# Autodesk Inventor assembly: AssembledCube
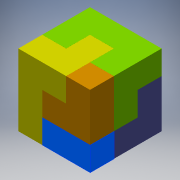
[picture p0: Inventor's stored thumbnail of the model, 180x180]
Saved by Autodesk Inventor 2019 (Build 230136000, 136)
## iProperties
Created: 2018-12-10
Part Number: AssembledCube
Document SubType Name: Assembly
Designer: Mihir
Author: Mihir
## Documents named in this file (6)
- C:\Users\Mihir\Documents\Inventor\AssembledCube.iam
- C:\Users\Mihir\Documents\Inventor\BluePiece.ipt
- C:\Users\Mihir\Documents\Inventor\GreenPiece.ipt
- C:\Users\Mihir\Documents\Inventor\OrangePiece.ipt
- C:\Users\Mihir\Documents\Inventor\PurplePiece.ipt
- C:\Users\Mihir\Documents\Inventor\YellowPiece.ipt
## Components (5 placed, 5 different names)
1. BluePiece:1 — Mate:2, Flush:3, Flush:4, Mate:3, Mate:4, Mate:7
2. GreenPiece:1 — Mate:6, Flush:6, Flush:7
3. OrangePiece:1 — Mate:1, Flush:1, Flush:2, Flush:5, Mate:5, Flush:7
4. PurplePiece:1 — Mate:1, Flush:1, Flush:2, Mate:2, Flush:3, Flush:4, Mate:6, Flush:6
5. YellowPiece:1 — Mate:3, Mate:4, Flush:5, Mate:5, Mate:7
## Relationships (14: Mate 7, Flush 7)
- Mate:1: OrangePiece:1 ↔ PurplePiece:1
- Flush:1: OrangePiece:1 ↔ PurplePiece:1
- Flush:2: OrangePiece:1 ↔ PurplePiece:1
- Mate:2: BluePiece:1 ↔ PurplePiece:1
- Flush:3: BluePiece:1 ↔ PurplePiece:1
- Flush:4: BluePiece:1 ↔ PurplePiece:1
- Mate:3: BluePiece:1 ↔ YellowPiece:1
- Mate:4: BluePiece:1 ↔ YellowPiece:1
- Flush:5: OrangePiece:1 ↔ YellowPiece:1
- Mate:5: OrangePiece:1 ↔ YellowPiece:1
- Mate:6: GreenPiece:1 ↔ PurplePiece:1
- Flush:6: GreenPiece:1 ↔ PurplePiece:1
- Flush:7: GreenPiece:1 ↔ OrangePiece:1
- Mate:7: BluePiece:1 ↔ YellowPiece:1
